# Autodesk Inventor assembly: 276-2181
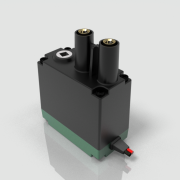
[picture p0: Inventor's stored thumbnail of the model, 180x180]
Saved by Autodesk Inventor 2015 SP1 (Build 190201100, 201)
## iProperties
Category: Motion
Company: Super Sonic Sparks, Team 24
Part Number: 276-2181
Document SubType Name: Assembly
Designer: Jordan Kiesel
Mass: 60.781 g
Surface Area: 280.554 cm^2
Volume: 17.9114 cm^3
Density: 3.39342 g/cm^3
Catalog Web Link: vexrobotics.com/276-2181.html
Description: Add motors to power more wheels or add an end effector.
Vendor: VEX Robotics, Inc.
Translation Standard: STEP AP203
FileName: 2-Wire Motor 269.iam
PreProcessor: SolidWorks 2009
PostProcessor: Build: 239, Release: 2011 RTM - Date: Wed 02/17/2010
Sent Units: inch
Uncertainty: 1e-05
Author: Jordan Kiesel
Title: 2-Wire Motor 269
Comments: Add motors to power more wheels or add an end effector to take your robot to the next level. ▷ Strong, steel internal gears. ▷ No clutches needed. ▷ Shaft coupler (included) replaces the clutch. ▷ Similar torque and speed to the 3-wire VEX Motor. ▷ The 2-Wire Motor 269 does not have an internal motor controller. The motor connects directly to 2-Wire Motor Ports (Ports 1 & 10 on the Cortex Microcontroller). For 3-Wire Motor Ports (Ports 2-9 on the Cortex), a Motor Controller 29 must be used in between the Microcontroller and the motor.
## Documents named in this file (19)
- C:\Users\Jordan\Documents\Robotics\VEX\CAD\2015 BNS CAD Library (beta)\Motion\Motors\2-Wire Motor 269.iam
- C:\Users\Jordan\Documents\Robotics\VEX\CAD\2015 BNS CAD Library (beta)\Motion\Motors\Reference Parts\2-Wire Motors\0.589'' Screw.ipt
- C:\Users\Jordan\Documents\Robotics\VEX\CAD\2015 BNS CAD Library (beta)\Motion\Motors\Reference Parts\2-Wire Motor 269\Top Housing.ipt
- C:\Users\Jordan\Documents\Robotics\VEX\CAD\2015 BNS CAD Library (beta)\Motion\Motors\Reference Parts\2-Wire Motors\6-32 Screw Insert Nut.ipt
- C:\Users\Jordan\Documents\Robotics\VEX\CAD\2015 BNS CAD Library (beta)\Motion\Motors\Reference Parts\2-Wire Motor 269\Bearing.ipt
- C:\Users\Jordan\Documents\Robotics\VEX\CAD\2015 BNS CAD Library (beta)\Motion\Motors\Reference Parts\2-Wire Motor 269\Internal Motor.ipt
- C:\Users\Jordan\Documents\Robotics\VEX\CAD\2015 BNS CAD Library (beta)\Motion\Motors\Reference Parts\2-Wire Motor 269\0.197'' Screw.ipt
- C:\Users\Jordan\Documents\Robotics\VEX\CAD\2015 BNS CAD Library (beta)\Motion\Motors\Reference Parts\2-Wire Motor 269\0.63'' Shaft.ipt
- C:\Users\Jordan\Documents\Robotics\VEX\CAD\2015 BNS CAD Library (beta)\Motion\Motors\Reference Parts\2-Wire Motor 269\Bottom Plate.ipt
- C:\Users\Jordan\Documents\Robotics\VEX\CAD\2015 BNS CAD Library (beta)\Motion\Motors\Reference Parts\2-Wire Motor 269\10-34-tooth Compound Gear.ipt
- C:\Users\Jordan\Documents\Robotics\VEX\CAD\2015 BNS CAD Library (beta)\Motion\Motors\Reference Parts\2-Wire Motor 269\10-34-tooth Long Compound Gear.ipt
- C:\Users\Jordan\Documents\Robotics\VEX\CAD\2015 BNS CAD Library (beta)\Motion\Motors\Reference Parts\Motors\2-Wire Cable Support.ipt
- C:\Users\Jordan\Documents\Robotics\VEX\CAD\2015 BNS CAD Library (beta)\Motion\Motors\Reference Parts\2-Wire Motor 269\Bottom Housing.ipt
- C:\Users\Jordan\Documents\Robotics\VEX\CAD\2015 BNS CAD Library (beta)\Motion\Motors\Reference Parts\2-Wire Motor 269\1.299'' Shaft.ipt
- C:\Users\Jordan\Documents\Robotics\VEX\CAD\2015 BNS CAD Library (beta)\Motion\Motors\Reference Parts\2-Wire Motor 269\10-tooth Input Gear.ipt
- C:\Users\Jordan\Documents\Robotics\VEX\CAD\2015 BNS CAD Library (beta)\Motion\Motors\Reference Parts\2-Wire Motor 269\10-24-tooth Compound Gear.ipt
- C:\Users\Jordan\Documents\Robotics\VEX\CAD\2015 BNS CAD Library (beta)\Motion\Motors\Reference Parts\2-Wire Motor 269\26-tooth Output Gear.ipt
- C:\Users\Jordan\Documents\Robotics\VEX\CAD\2015 BNS CAD Library (beta)\Motion\Motors\Reference Parts\2-Wire Motor 269\Internal Motor Carrier.ipt
- C:\Users\Jordan\Documents\Robotics\VEX\CAD\2015 BNS CAD Library (beta)\Motion\Motors\Reference Parts\2-Wire Motors\2-Wire Motor Cable, Cut.ipt
## Components (30 placed, 18 different names)
1. 0.589'' Screw:1 — Insert:23
2. Top Housing:1 — Insert:1, Insert:2, Insert:3, Insert:4, Insert:5, Insert:6, Insert:7, Insert:8, Insert:9, Insert:11, Insert:12
3. 6-32 Screw Insert Nut:1 — Insert:8
4. Bearing:1 — Insert:21, Insert:22
5. 2-Wire Motor Cable, Cut:1
6. Internal Motor:1 — Angle:1, Insert:10, Insert:13
7. 0.197'' Screw:1 — Insert:18
8. 0.63'' Shaft:1 — Insert:19
9. Bottom Plate:1 — Insert:23, Insert:24, Insert:25, Insert:26, Insert:27, Insert:28
10. 10-34-tooth Compound Gear:1 — Insert:20, Rotation:2, Rotation:3
11. 10-34-tooth Long Compound Gear:1 — Insert:12, Insert:14, Rotation:1, Rotation:2
12. 0.63'' Shaft:2 — Insert:15
13. 2-Wire Cable Support:1
14. 10-34-tooth Compound Gear:2 — Insert:14, Rotation:3, Rotation:4
15. Bottom Housing:1 — Insert:6, Insert:7, Insert:15, Insert:16, Insert:17, Insert:18, Insert:19, Insert:20, Insert:21, Insert:27, Insert:28
16. 1.299'' Shaft:1 — Insert:11
17. 0.589'' Screw:2 — Insert:2
18. Bearing:2 — Insert:9
19. 6-32 Screw Insert Nut:2 — Insert:5
20. 0.589'' Screw:3 — Insert:25
21. 0.589'' Screw:4 — Insert:3
22. 0.589'' Screw:5 — Insert:26
23. 0.589'' Screw:6 — Insert:4
24. 0.589'' Screw:7 — Insert:24
25. 0.589'' Screw:8 — Insert:1
26. 0.197'' Screw:2 — Insert:17
27. 10-tooth Input Gear:1 — Insert:13, Rotation:5
28. 10-24-tooth Compound Gear:1 — Insert:16, Rotation:4, Rotation:5
29. 26-tooth Output Gear:1 — Insert:22, Rotation:1
30. Internal Motor Carrier:1 — Angle:1, Insert:10
## Relationships (34: Insert 28, RelateRotation 5, Angle 1)
- Insert:1: Top Housing:1 ↔ 0.589'' Screw:8
- Insert:2: Top Housing:1 ↔ 0.589'' Screw:2
- Insert:3: Top Housing:1 ↔ 0.589'' Screw:4
- Insert:4: Top Housing:1 ↔ 0.589'' Screw:6
- Insert:5: Top Housing:1 ↔ 6-32 Screw Insert Nut:2
- Insert:6: Top Housing:1 ↔ Bottom Housing:1
- Insert:7: Top Housing:1 ↔ Bottom Housing:1
- Insert:8: Top Housing:1 ↔ 6-32 Screw Insert Nut:1
- Insert:9: Top Housing:1 ↔ Bearing:2
- Angle:1 (0 deg): Internal Motor:1 ↔ Internal Motor Carrier:1
- Insert:10: Internal Motor:1 ↔ Internal Motor Carrier:1
- Insert:11: Top Housing:1 ↔ 1.299'' Shaft:1
- Insert:12 (0.1016 mm): Top Housing:1 ↔ 10-34-tooth Long Compound Gear:1
- Insert:13 (0.889 mm): Internal Motor:1 ↔ 10-tooth Input Gear:1
- Insert:14: 10-34-tooth Long Compound Gear:1 ↔ 10-34-tooth Compound Gear:2
- Insert:15: 0.63'' Shaft:2 ↔ Bottom Housing:1
- Insert:16: Bottom Housing:1 ↔ 10-24-tooth Compound Gear:1
- Insert:17: Bottom Housing:1 ↔ 0.197'' Screw:2
- Insert:18: 0.197'' Screw:1 ↔ Bottom Housing:1
- Insert:19: 0.63'' Shaft:1 ↔ Bottom Housing:1
- Insert:20: 10-34-tooth Compound Gear:1 ↔ Bottom Housing:1
- Insert:21 (0.1016 mm): Bearing:1 ↔ Bottom Housing:1
- Insert:22: Bearing:1 ↔ 26-tooth Output Gear:1
- Insert:23: 0.589'' Screw:1 ↔ Bottom Plate:1
- Insert:24: Bottom Plate:1 ↔ 0.589'' Screw:7
- Insert:25: Bottom Plate:1 ↔ 0.589'' Screw:3
- Insert:26: Bottom Plate:1 ↔ 0.589'' Screw:5
- Insert:27: Bottom Plate:1 ↔ Bottom Housing:1
- Insert:28: Bottom Plate:1 ↔ Bottom Housing:1
- Rotation:1 [RelateRotation] (2.6 ul): 10-34-tooth Long Compound Gear:1 ↔ 26-tooth Output Gear:1
- Rotation:2 [RelateRotation] (3.4 ul): 10-34-tooth Compound Gear:1 ↔ 10-34-tooth Long Compound Gear:1
- Rotation:3 [RelateRotation] (3.4 ul): 10-34-tooth Compound Gear:1 ↔ 10-34-tooth Compound Gear:2
- Rotation:4 [RelateRotation] (3.4 ul): 10-34-tooth Compound Gear:2 ↔ 10-24-tooth Compound Gear:1
- Rotation:5 [RelateRotation] (2.4 ul): 10-tooth Input Gear:1 ↔ 10-24-tooth Compound Gear:1
